# Autodesk Inventor assembly: AM Shifter Cluster Shaft subassembly
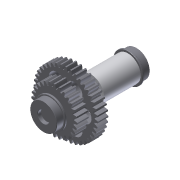
[picture p0: Inventor's stored thumbnail of the model, 180x180]
Saved by Autodesk Inventor 2011 (Build 150239000, 239)
## iProperties
Created: 2012-06-03
Part Number: AM Shifter Cluster Shaft subassembly
Document SubType Name: Assembly
Designer: Nemo
Author: Nemo
## Documents named in this file (7)
- H:\Nemo\Documents\Robotics\COTS Parts\Gearboxes\Shafts\AM Shifter Cluster Shaft subassembly.iam
- H:\Nemo\Documents\Robotics\COTS Parts\Gearboxes\Shafts\AM Shifter Cluster Shaft.ipt
- H:\Nemo\Documents\Robotics\COTS Parts\Gearboxes\Bearings\Bearing FR6zz.ipt
- H:\Nemo\Documents\Robotics\COTS Parts\Gearboxes\Gears\Gear 20dp 375hex 40T.ipt
- H:\Nemo\Documents\Robotics\COTS Parts\Gearboxes\Gears\Gear 20dp 375hex 15T.ipt
- H:\Nemo\Documents\Robotics\COTS Parts\Gearboxes\Gears\Gear 20dp 375hex 28T.ipt
- H:\Nemo\Documents\Robotics\COTS Parts\Gearboxes\Spacers\AM Shifter cluster spacer.ipt
## Components (7 placed, 6 different names)
1. AM Shifter Cluster Shaft:1 — Insert:1, Insert:2, Mate:1, Mate:2, Mate:3, Angle:1, Angle:2, Angle:3
2. Bearing FR6zz:1 — Insert:2, Mate:7, Mate:8
3. Bearing FR6zz:2 — Insert:1, Mate:9
4. Gear 40T 20dp 375hex:1 — Mate:2, Angle:1, Mate:4, Mate:5
5. Gear 15T 20dp 375hex:1 — Mate:3, Angle:3, Mate:5
6. Gear 28T 20dp 375 hex:1 — Mate:1, Angle:2, Mate:4, Mate:9
7. AM Shifter cluster spacer:1 — Mate:7, Mate:8
## Relationships (13: Mate 8, Angle 3, Insert 2)
- Insert:1: AM Shifter Cluster Shaft:1 ↔ Bearing FR6zz:2
- Insert:2: AM Shifter Cluster Shaft:1 ↔ Bearing FR6zz:1
- Mate:1: AM Shifter Cluster Shaft:1 ↔ Gear 28T 20dp 375 hex:1
- Mate:2: AM Shifter Cluster Shaft:1 ↔ Gear 40T 20dp 375hex:1
- Mate:3: AM Shifter Cluster Shaft:1 ↔ Gear 15T 20dp 375hex:1
- Angle:1 (0 deg): AM Shifter Cluster Shaft:1 ↔ Gear 40T 20dp 375hex:1
- Angle:2 (0 deg): AM Shifter Cluster Shaft:1 ↔ Gear 28T 20dp 375 hex:1
- Angle:3 (0 deg): AM Shifter Cluster Shaft:1 ↔ Gear 15T 20dp 375hex:1
- Mate:4: Gear 40T 20dp 375hex:1 ↔ Gear 28T 20dp 375 hex:1
- Mate:5: Gear 40T 20dp 375hex:1 ↔ Gear 15T 20dp 375hex:1
- Mate:7 (0.0508 mm): Bearing FR6zz:1 ↔ AM Shifter cluster spacer:1
- Mate:8: Bearing FR6zz:1 ↔ AM Shifter cluster spacer:1
- Mate:9 (1.8034 mm): Bearing FR6zz:2 ↔ Gear 28T 20dp 375 hex:1
